# Autodesk Inventor assembly: LAIRD_001-0012
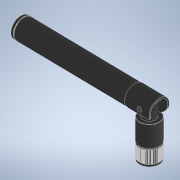
[picture p0: Inventor's stored thumbnail of the model, 180x180]
Saved by Autodesk Inventor 2021 (Build 250183000, 183)
## iProperties
Created: 2020-06-10
Part Number: LAIRD_001-0012
Document SubType Name: Assembly
Designer: lgnds
Author: lgnds
## Documents named in this file (3)
- C:\Users\lgnds\Google Drive\Unicorn 2020\CAD\WIFI\LAIRD_001-0012.iam
- C:\Users\lgnds\Google Drive\Unicorn 2020\CAD\WIFI\LAIRD_001-0012_Lower.ipt
- C:\Users\lgnds\Google Drive\Unicorn 2020\CAD\WIFI\LAIRD_001-0012_Upper.ipt
## Components (2 placed, 2 different names)
1. LAIRD_001-0012_Lower:1 — Rotational:1
2. LAIRD_001-0012_Upper:1 — Rotational:1
## Relationships (1: RevoluteJoint 1)
- Rotational:1 [RevoluteJoint]: LAIRD_001-0012_Lower:1 ↔ LAIRD_001-0012_Upper:1
